# Autodesk Inventor assembly: 8B
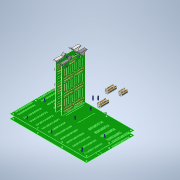
[picture p0: Inventor's stored thumbnail of the model, 180x180]
Saved by Autodesk Inventor 2021 (Build 250183000, 183)
## iProperties
Created: 2022-07-03
Part Number: 8B
Document SubType Name: Assembly
Designer: erics
Author: erics
## Documents named in this file (5)
- D:\Users\erics\Documents\16B\Mechanical\8B.iam
- D:\Users\erics\Documents\16B\Backplane\Mechanical\Backplane.iam
- D:\Users\erics\Documents\16B\Scratch\Mechanical\Scratch.iam
- D:\Users\erics\Documents\16B\Control Logic\Mechanical\Control Logic.iam
- D:\Users\erics\Documents\16B\Register\Mechanical\Register.iam
## Components (4 placed, 4 different names)
1. Backplane:1 [sub-assembly] — Flush:1, Flush:2, Mate:1, Flush:3
2. Scratch:1 [sub-assembly] — Flush:3, Angle:1, Mate:2, Mate:3
3. Control Logic:1 [sub-assembly] — Flush:5, Mate:4, Flush:8
4. Register:1 [sub-assembly] — Angle:2, Mate:5, Flush:9, Mate:6
## Relationships (14: Flush 6, Mate 6, Angle 2)
- Flush:1: Backplane:1
- Flush:2: Backplane:1
- Mate:1: Backplane:1
- Flush:3 (19.05 mm): Backplane:1 ↔ Scratch:1
- Angle:1 (180 deg): Scratch:1
- Mate:2 (-63.5 mm): Scratch:1
- Mate:3 (112.96 mm): Scratch:1
- Flush:5: Control Logic:1
- Mate:4: Control Logic:1
- Flush:8 (12.7 mm): Control Logic:1
- Angle:2 (180 deg): Register:1
- Mate:5 (95.18 mm): Register:1
- Flush:9 (19.05 mm): Register:1
- Mate:6 (-63.5 mm): Register:1
## Named parameters: CCA_Offset = 6.35 mm, Row_Offset = -63.5 mm
